# Autodesk Inventor assembly: F-Upright20181
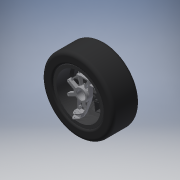
[picture p0: Inventor's stored thumbnail of the model, 180x180]
Saved by Autodesk Inventor 2018.2 (Build 222227000, 227)
## iProperties
Created: 2018-05-19
Part Number: F-Upright20181
Material: 一般
Document SubType Name: Assembly
Designer: ku_sk
Sending System: Autodesk Inventor 2018
Preprocessor: ST-DEVELOPER v17
Title: D:\ku_sk\ドキュメント\Inventor\Aero\KS-15\全体アッセンブリ解析用モデル\body\sus\F-Upright2018.stp
Author: ku_sk
## Documents named in this file (5)
- D:\ku_sk\ドキュメント\Inventor\Aero\KS-15\全体アッセンブリ解析用モデル\body\sus\F-Upright20181.iam
- D:\ku_sk\ドキュメント\Inventor\Aero\KS-15\全体アッセンブリ解析用モデル\body\sus\Part31.ipt
- D:\ku_sk\ドキュメント\Inventor\Aero\KS-15\全体アッセンブリ解析用モデル\body\sus\Part41.ipt
- D:\ku_sk\ドキュメント\Inventor\Aero\KS-15\全体アッセンブリ解析用モデル\body\sus\Part21.ipt
- D:\ku_sk\ドキュメント\Inventor\Aero\KS-15\全体アッセンブリ解析用モデル\body\sus\2015Wheel watanabe1.ipt
## Components (4 placed, 4 different names)
1. Part31:1 — メイト:2, メイト:1
2. Part41:1
3. Part21:1
4. 2015Wheel watanabe1:1 — メイト:2, メイト:1
## Relationships (2: Mate 2)
- メイト:2 [Mate] (49 mm): Part31:1 ↔ 2015Wheel watanabe1:1
- メイト:1 [Mate]: Part31:1 ↔ 2015Wheel watanabe1:1
